# Autodesk Inventor assembly: mountedLifterMotor
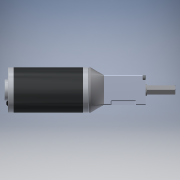
[picture p0: Inventor's stored thumbnail of the model, 180x180]
Saved by Autodesk Inventor 2017 (Build 210142000, 142)
## iProperties
Created: 2017-03-08
Part Number: mountedLifterMotor
Document SubType Name: Assembly
Designer: kingb
Author: kingb
## Documents named in this file (9)
- C:\Users\kingb\Desktop\CAD\mountedLifterMotor.iam
- C:\Users\kingb\Desktop\CAD\217-2625-001 Rev1.ipt
- C:\Users\kingb\Desktop\CAD\217-2625-002 Rev1.ipt
- C:\Users\kingb\Desktop\CAD\217-2816-001 Rev1.ipt
- C:\Users\kingb\Desktop\CAD\217-4018-STEP-20140806.ipt
- C:\Users\kingb\Desktop\CAD\SSA_SSA0832-1750ZC.ipt
- C:\Users\kingb\Desktop\CAD\25inCIM.ipt
- C:\Users\kingb\Desktop\CAD\10-32x0500_shcs_HX-SHCS 0.19-32x1.375x1-C.ipt
- C:\Users\kingb\Desktop\CAD\217-2897.20121205.ipt
## Components (11 placed, 8 different names)
1. 217-2625-001 Rev1:1 — Insert:1, Insert:2, Mate:1, Mate:2, Mate:3
2. 217-2625-002 Rev1:1 — Insert:5, Insert:6, Insert:7, Insert:8, Mate:6, Mate:7
3. 217-2816-001 Rev1:1 — Insert:1, Insert:2, Insert:3, Insert:4
4. 217-2816-001 Rev1:2 — Insert:3, Insert:4, Insert:5, Insert:6
5. 217-4018-STEP-20140806:1 — Mate:1, Mate:2, Mate:3, Insert:10, Insert:11, Insert:12
6. SSA_SSA0832-1750ZC:1 — Insert:8
7. SSA_SSA0832-1750ZC:2 — Insert:7
8. 25inCIM:1 — Mate:4, Mate:5, Insert:12
9. 10-32x0500_shcs_HX-SHCS 0.19-32x1.375x1-C:1 — Insert:10, Mate:5
10. 10-32x0500_shcs_HX-SHCS 0.19-32x1.375x1-C:2 — Insert:11, Mate:4
11. 217-2897.20121205:1 — Mate:6, Mate:7
## Relationships (18: Insert 11, Mate 7)
- Insert:1: 217-2625-001 Rev1:1 ↔ 217-2816-001 Rev1:1
- Insert:2: 217-2625-001 Rev1:1 ↔ 217-2816-001 Rev1:1
- Insert:3: 217-2816-001 Rev1:1 ↔ 217-2816-001 Rev1:2
- Insert:4: 217-2816-001 Rev1:1 ↔ 217-2816-001 Rev1:2
- Insert:5: 217-2625-002 Rev1:1 ↔ 217-2816-001 Rev1:2
- Insert:6: 217-2625-002 Rev1:1 ↔ 217-2816-001 Rev1:2
- Mate:1: 217-2625-001 Rev1:1 ↔ 217-4018-STEP-20140806:1
- Mate:2: 217-2625-001 Rev1:1 ↔ 217-4018-STEP-20140806:1
- Mate:3: 217-2625-001 Rev1:1 ↔ 217-4018-STEP-20140806:1
- Insert:7: 217-2625-002 Rev1:1 ↔ SSA_SSA0832-1750ZC:2
- Insert:8: 217-2625-002 Rev1:1 ↔ SSA_SSA0832-1750ZC:1
- Insert:10: 217-4018-STEP-20140806:1 ↔ 10-32x0500_shcs_HX-SHCS 0.19-32x1.375x1-C:1
- Insert:11: 217-4018-STEP-20140806:1 ↔ 10-32x0500_shcs_HX-SHCS 0.19-32x1.375x1-C:2
- Mate:4: 25inCIM:1 ↔ 10-32x0500_shcs_HX-SHCS 0.19-32x1.375x1-C:2
- Mate:5: 25inCIM:1 ↔ 10-32x0500_shcs_HX-SHCS 0.19-32x1.375x1-C:1
- Insert:12: 217-4018-STEP-20140806:1 ↔ 25inCIM:1
- Mate:6: 217-2625-002 Rev1:1 ↔ 217-2897.20121205:1
- Mate:7: 217-2625-002 Rev1:1 ↔ 217-2897.20121205:1
